# Autodesk Inventor assembly: ASY GBK bottom 0020
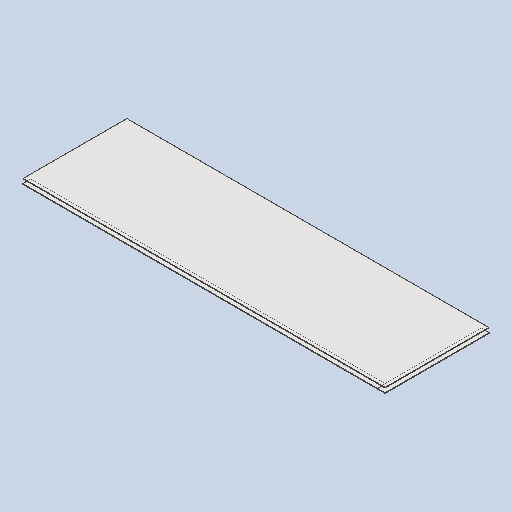
[picture p0: Inventor's stored thumbnail of the model, 512x512]
Saved by Autodesk Inventor 2026.3 (Build 303398000, 398)
## iProperties
Created: 2026-07-15
Part Number: ASY GBK bottom 0020
Document SubType Name: Assembly
Designer: admin
Mass: 109378 g
Surface Area: 56508.2 cm^2
Volume: 13933.6 cm^3
Density: 7.85 g/cm^3
Stock Number: 0020
Author: admin
## Documents named in this file (4)
- C:\Users\admin\Documents\Inventor\GBK-Gubkinskiy\ASY GBK bottom 0020.iam
- C:\Users\admin\Documents\Inventor\GBK-Gubkinskiy\Пол\GBK bottom 0112.ipt
- C:\Users\admin\Documents\Inventor\GBK-Gubkinskiy\Пол\GBK bottom 0135.ipt
- C:\Users\admin\Documents\Inventor\GBK-Gubkinskiy\Пол\GBK bottom 0132.ipt
## Components (3 placed, 3 different names)
1. GBK bottom 0112:1
2. GBK bottom 0135:1
3. GBK bottom 0132:1
## Relationships (4: Mate 3, WeldJoint 1)
- [WeldJoint]: GBK bottom 0135:1 ↔ GBK bottom 0132:1
- [Mate]: GBK bottom 0112:1 ↔ GBK bottom 0132:1
- [Mate] (-30 mm): GBK bottom 0112:1 ↔ GBK bottom 0135:1
- [Mate] (-30 mm): GBK bottom 0112:1 ↔ GBK bottom 0132:1
